# Autodesk Inventor assembly: B Drive
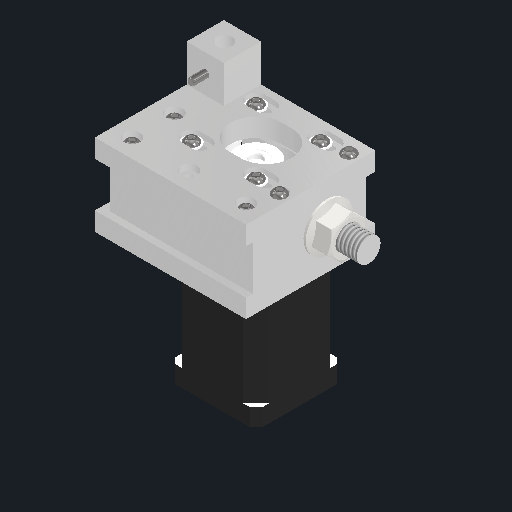
[picture p0: Inventor's stored thumbnail of the model, 512x512]
Saved by Autodesk Inventor 2025.1 (Build 291241020, 241B)
## iProperties
Created: 2025-05-09
Part Number: B Drive
Document SubType Name: Assembly
Designer: AdminForWorker
Title: B Drive
Author: AdminForWorker
## Documents named in this file (4)
- C:\Users\Joshua Eah\Documents\Voron 0.2\CAD\Master Assembly\B Drive.iam
- C:\Users\Joshua Eah\Documents\Voron 0.2\CAD\Master Assembly\Motor Assembly (1).iam
- C:\Users\Joshua Eah\Documents\Voron 0.2\CAD\Machined Parts\AB Drives\B Drive\B Drive Assembly.iam
- C:\Users\Joshua Eah\Documents\Voron 0.2\CAD\Master Assembly\Hardware\Hardware Assemblies\Hardware (8).iam
## Components (3 placed, 3 different names)
1. Motor Assembly (1):1 [sub-assembly]
2. B Drive Assembly:1 [sub-assembly] — Insert:1, Insert:2
3. Hardware (8):1 [sub-assembly] — Insert:1, Insert:2
## Relationships (2: Insert 2)
- Insert:1: B Drive Assembly:1 ↔ Hardware (8):1
- Insert:2: B Drive Assembly:1 ↔ Hardware (8):1
